# Autodesk Inventor assembly: サス
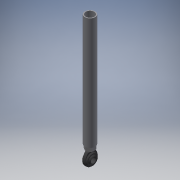
[picture p0: Inventor's stored thumbnail of the model, 180x180]
Saved by Autodesk Inventor 2018 (Build 220112000, 112)
## iProperties
Created: 2017-09-07
Part Number: サス
Material: 一般
Document SubType Name: Assembly
Designer: Kosei
Author: Kosei
## Documents named in this file (5)
- C:\Users\mura5\Documents\RBBR\cart\サス.iam
- C:\Users\mura5\Documents\RBBR\cart\Part1.ipt
- C:\Users\mura5\Documents\RBBR\cart\Pipe1.ipt
- C:\Users\mura5\Documents\RBBR\cart\hn1_14.ipt
- C:\Users\mura5\Documents\RBBR\cart\iko_POS_14EC\AIS2016\POS 14EC.iam
## Components (4 placed, 4 different names)
1. Part1:1
2. Pipe1:1 — リジッド:2
3. hn1_14:2 — リジッド:2, リジッド:3
4. POS 14EC:1 [sub-assembly] — リジッド:3
## Relationships (2: WeldJoint 2)
- リジッド:2 [WeldJoint]: Pipe1:1 ↔ hn1_14:2
- リジッド:3 [WeldJoint]: hn1_14:2 ↔ POS 14EC:1
